# Autodesk Inventor assembly: hv_transformer
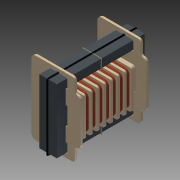
[picture p0: Inventor's stored thumbnail of the model, 180x180]
Saved by Autodesk Inventor 2015 (Build 190159000, 159)
## iProperties
Created: 2014-10-08
Part Number: hv_transformer
Document SubType Name: Assembly
Designer: Adam
Author: Adam
## Documents named in this file (6)
- C:\Users\nopassword\Desktop\AX100\Assembly\hv_transformer.iam
- C:\Users\nopassword\Desktop\AX100\Assembly\hv_x-former_bobbin.ipt
- C:\Users\nopassword\Desktop\AX100\Assembly\leakage.ipt
- C:\Users\nopassword\Desktop\AX100\Assembly\TSC_EL375.ipt
- C:\Users\nopassword\Desktop\AX100\Assembly\twine.ipt
- C:\Users\nopassword\Desktop\AX100\Assembly\wire.ipt
## Components (6 placed, 5 different names)
1. hv_x-former_bobbin:1 — Mate:3, Mate:4, Mate:5, Flush:8, Mate:7, Mate:8
2. leakage:1 — Mate:1, Flush:1, Flush:2, Mate:2
3. TSC_EL375:1 — Mate:2, Flush:3, Flush:4, Flush:5, Flush:7
4. twine:1 — Flush:5, Flush:7, Mate:6
5. wire:1 — Flush:8, Mate:7, Tangent:2
6. TSC_EL375:2 — Mate:1, Flush:1, Flush:2, Flush:3, Flush:4, Mate:3, Mate:4, Mate:5, Mate:6
## Relationships (16: Mate 8, Flush 7, Tangent 1)
- Mate:1: leakage:1 ↔ TSC_EL375:2
- Flush:1 (0.5 mm): leakage:1 ↔ TSC_EL375:2
- Flush:2 (0.5 mm): leakage:1 ↔ TSC_EL375:2
- Mate:2: leakage:1 ↔ TSC_EL375:1
- Flush:3: TSC_EL375:1 ↔ TSC_EL375:2
- Flush:4: TSC_EL375:1 ↔ TSC_EL375:2
- Mate:3 (0.5 mm): hv_x-former_bobbin:1 ↔ TSC_EL375:2
- Mate:4 (0.5 mm): hv_x-former_bobbin:1 ↔ TSC_EL375:2
- Mate:5 (0.5 mm): hv_x-former_bobbin:1 ↔ TSC_EL375:2
- Flush:5: TSC_EL375:1 ↔ twine:1
- Flush:7 (0.25 mm): TSC_EL375:1 ↔ twine:1
- Mate:6: twine:1 ↔ TSC_EL375:2
- Flush:8: hv_x-former_bobbin:1 ↔ wire:1
- Mate:7: hv_x-former_bobbin:1 ↔ wire:1
- Tangent:2: wire:1
- Mate:8: hv_x-former_bobbin:1
